# Autodesk Inventor assembly: BC-100000-Inf
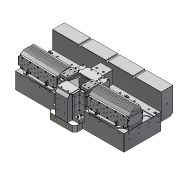
[picture p0: Inventor's stored thumbnail of the model, 180x180]
Saved by Autodesk Inventor 2016 (Build 200138000, 138)
## iProperties
Created: 2015-09-16
Part Number: BC-100000-Inf
Document SubType Name: Assembly
Designer: Reinaldo.Basílio
Mass: 576635 g
Surface Area: 46856.4 cm^2
Volume: 76554.8 cm^3
Density: 7.53231 g/cm^3
Author: Reinaldo.Basílio
## Documents named in this file (40)
- D:\ARQ\Basilio\LNLS-2\Anel\Dipolos\BC-3T\Dipolo 3T e 1T\Prototipo 1\Projeto Mecanico\BC-100000-Inf.iam
- D:\ARQ\Basilio\LNLS-2\Anel\Dipolos\BC-3T\Dipolo 3T e 1T\Prototipo 1\Projeto Mecanico\BC-100004.iam
- D:\ARQ\Basilio\LNLS-2\Anel\Dipolos\BC-3T\Dipolo 3T e 1T\Prototipo 1\Projeto Mecanico\BC-10005.ipt
- D:\ARQ\Basilio\LNLS-2\Anel\Dipolos\BC-3T\Dipolo 3T e 1T\Prototipo 1\Projeto Mecanico\BC-100005.iam
- D:\ARQ\Basilio\LNLS-2\Anel\Dipolos\BC-3T\Dipolo 3T e 1T\Prototipo 1\Projeto Mecanico\BC-10008.ipt
- D:\ARQ\Basilio\LNLS-2\Anel\Dipolos\BC-3T\Dipolo 3T e 1T\Prototipo 1\Projeto Mecanico\BC-10007.ipt
- D:\ARQ\Basilio\LNLS-2\Anel\Dipolos\BC-3T\Dipolo 3T e 1T\Prototipo 1\Projeto Mecanico\BC-10001.ipt
- D:\ARQ\Basilio\LNLS-2\Anel\Dipolos\BC-3T\Dipolo 3T e 1T\Prototipo 1\Projeto Mecanico\BC-10019-A.ipt
- D:\ARQ\Basilio\LNLS-2\Anel\Dipolos\BC-3T\Dipolo 3T e 1T\Prototipo 1\Projeto Mecanico\BC-100001-A-Inf.iam
- D:\ARQ\Basilio\LNLS-2\Anel\Dipolos\BC-3T\Dipolo 3T e 1T\Prototipo 1\Projeto Mecanico\BC-10002.ipt
- D:\ARQ\Basilio\LNLS-2\Anel\Dipolos\BC-3T\Dipolo 3T e 1T\Prototipo 1\Projeto Mecanico\BC-10006.ipt
- D:\ARQ\Basilio\LNLS-2\Anel\Dipolos\BC-3T\Dipolo 3T e 1T\Prototipo 1\Projeto Mecanico\BC-100001-B-Inf.iam
- D:\ARQ\Basilio\LNLS-2\Anel\Dipolos\BC-3T\Dipolo 3T e 1T\Prototipo 1\Projeto Mecanico\BC-10011.ipt
- D:\ARQ\Basilio\LNLS-2\Anel\Dipolos\BC-3T\Dipolo 3T e 1T\Prototipo 1\Projeto Mecanico\BC-10012.ipt
- D:\ARQ\Basilio\LNLS-2\Anel\Dipolos\BC-3T\Dipolo 3T e 1T\Prototipo 1\Projeto Mecanico\BC-10013.ipt
- D:\ARQ\Basilio\LNLS-2\Anel\Dipolos\BC-3T\Dipolo 3T e 1T\Prototipo 1\Projeto Mecanico\BC-10014.ipt
- D:\ARQ\Basilio\LNLS-2\Anel\Dipolos\BC-3T\Dipolo 3T e 1T\Prototipo 1\Projeto Mecanico\BC-10019-B.ipt
- D:\ARQ\Basilio\LNLS-2\Anel\Dipolos\BC-3T\Dipolo 3T e 1T\Prototipo 1\Projeto Mecanico\BC-10015.ipt
- D:\ARQ\Basilio\LNLS-2\Anel\Dipolos\BC-3T\Dipolo 3T e 1T\Prototipo 1\Projeto Mecanico\BC-10016.ipt
- D:\ARQ\Basilio\LNLS-2\Anel\Dipolos\BC-3T\Dipolo 3T e 1T\Prototipo 1\Projeto Mecanico\BC-10021.ipt
- D:\ARQ\Basilio\LNLS-2\Anel\Dipolos\BC-3T\Dipolo 3T e 1T\Prototipo 1\Projeto Mecanico\BC-10022.ipt
- D:\ARQ\Basilio\LNLS-2\Anel\Dipolos\BC-3T\Dipolo 3T e 1T\Prototipo 1\Projeto Mecanico\BC-10023.ipt
- D:\ARQ\Basilio\LNLS-2\Anel\Dipolos\BC-3T\Dipolo 3T e 1T\Prototipo 1\Projeto Mecanico\BC-10025.ipt
- D:\ARQ\Basilio\LNLS-2\Anel\Dipolos\BC-3T\Dipolo 3T e 1T\Prototipo 1\Projeto Mecanico\BC-10020.ipt
- D:\ARQ\Basilio\LNLS-2\Anel\Dipolos\BC-3T\Dipolo 3T e 1T\Prototipo 1\Projeto Mecanico\Parafusos\DIN 912 - M8x30.ipt
- D:\ARQ\Basilio\LNLS-2\Anel\Dipolos\BC-3T\Dipolo 3T e 1T\Prototipo 1\Projeto Mecanico\Parafusos\DIN 912 - M12x65.ipt
- D:\ARQ\Basilio\LNLS-2\Anel\Dipolos\BC-3T\Dipolo 3T e 1T\Prototipo 1\Projeto Mecanico\Parafusos\DIN 912 - M8x80.ipt
- D:\ARQ\Basilio\LNLS-2\Anel\Dipolos\BC-3T\Dipolo 3T e 1T\Prototipo 1\Projeto Mecanico\Parafusos\DIN 912 - M10x50.ipt
- D:\ARQ\Basilio\LNLS-2\Anel\Dipolos\BC-3T\Dipolo 3T e 1T\Prototipo 1\Projeto Mecanico\Parafusos\DIN 912 - M4x12.ipt
- D:\ARQ\Basilio\LNLS-2\Anel\Dipolos\BC-3T\Dipolo 3T e 1T\Prototipo 1\Projeto Mecanico\Parafusos\DIN 912 - M5x16.ipt
- D:\ARQ\Basilio\LNLS-2\Anel\Dipolos\BC-3T\Dipolo 3T e 1T\Prototipo 1\Projeto Mecanico\Parafusos\DIN 7991 - M5x12.ipt
- D:\ARQ\Basilio\LNLS-2\Anel\Dipolos\BC-3T\Dipolo 3T e 1T\Prototipo 1\Projeto Mecanico\Parafusos\DIN 125 - A 10,5.ipt
- D:\ARQ\Basilio\LNLS-2\Anel\Dipolos\BC-3T\Dipolo 3T e 1T\Prototipo 1\Projeto Mecanico\Parafusos\DIN 912 - M10x40.ipt
- D:\ARQ\Basilio\LNLS-2\Anel\Dipolos\BC-3T\Dipolo 3T e 1T\Prototipo 1\Projeto Mecanico\Parafusos\DIN 912 - M8x20.ipt
- D:\ARQ\Basilio\LNLS-2\Anel\Dipolos\BC-3T\Dipolo 3T e 1T\Prototipo 1\Projeto Mecanico\Parafusos\DIN 912 - M8x40.ipt
- D:\ARQ\Basilio\LNLS-2\Anel\Dipolos\BC-3T\Dipolo 3T e 1T\Prototipo 1\Projeto Mecanico\Parafusos\DIN 933 - M4x14.ipt
- D:\ARQ\Basilio\LNLS-2\Anel\Dipolos\BC-3T\Dipolo 3T e 1T\Prototipo 1\Projeto Mecanico\Parafusos\DIN 912 - M4x18.ipt
- D:\ARQ\Basilio\LNLS-2\Anel\Dipolos\BC-3T\Dipolo 3T e 1T\Prototipo 1\Projeto Mecanico\BC-10026.ipt
- D:\ARQ\Basilio\LNLS-2\Anel\Dipolos\BC-3T\Dipolo 3T e 1T\Prototipo 1\Projeto Mecanico\BC-10027.ipt
- D:\ARQ\Basilio\LNLS-2\Anel\Dipolos\BC-3T\Dipolo 3T e 1T\Prototipo 1\Projeto Mecanico\BC-100001\AIP\FEA\bjj5sjykh.fres
## Components (140 placed, 38 different names)
1. BC-10001:1 — Flush:41, Mate:39, Mate:48, Mate:50, Mate:52, Flush:57, Insert:3, Mate:53, Insert:6, Insert:7, Insert:8, Mate:54, Mate:55, Insert:13, Insert:15, Insert:16, Insert:22, Insert:23, Insert:24, Insert:25, Insert:26, Insert:27, Mate:57, Mate:62, Insert:30, Insert:31, Insert:48, Insert:49, Insert:50, Insert:51, Insert:52, Insert:53, Insert:54, Insert:55, Insert:56, Insert:57, Insert:58, Insert:59, Insert:154, Insert:155
2. BC-10002:1 — Flush:46, Mate:48, Mate:49, Insert:17, Insert:18, Insert:19, Insert:20, Insert:36, Insert:37, Insert:76, Insert:77
3. BC-10006:1 — Mate:52, Flush:57, Flush:58, Insert:68, Insert:69, Insert:70, Insert:71, Insert:72, Insert:73, Insert:74, Insert:75
4. BC-100005:1 [sub-assembly] — Flush:28, Mate:30, Flush:35, Mate:49, Mate:53
5. BC-100004:1 [sub-assembly] — Flush:24, Mate:17, Flush:25, Flush:26, Mate:50
6. BC-10019-B:1 — Insert:13, Insert:14, Insert:118, Insert:119, Insert:120, Insert:121
7. BC-10019-A:1 — Mate:39, Mate:40, Mate:41, Insert:110, Insert:111, Insert:112, Insert:113
8. BC-10005:1 — Mate:17, Flush:25, Flush:26, Mate:18, Flush:27, Flush:28, Mate:22, Flush:29, Mate:24, Flush:30, Mate:28, Flush:33, Mate:29, Flush:34, Mate:30, Flush:41, Mate:40, Mate:41, Flush:46, Insert:14
9. BC-100004:2 [sub-assembly] — Mate:22, Flush:29, Flush:31, Mate:59
10. BC-100004:3 [sub-assembly] — Mate:24, Flush:30, Flush:32, Flush:35, Mate:60
11. BC-100005:2 [sub-assembly] — Mate:18, Flush:27, Flush:31, Flush:32, Flush:34, Mate:61
12. BC-10008:1 — Insert:28, Insert:29, Insert:30, Insert:31, Insert:82, Insert:83, Insert:84, Insert:85
13. BC-10007:1 — Insert:28, Insert:29
14. BC-100001-A-Inf:1 [sub-assembly] — Insert:3, Tangent:2, Mate:54, Mate:63, Mate:64, Mate:65, Mate:66
15. BC-100001-B-Inf:1 [sub-assembly] — Insert:6, Tangent:1, Mate:55, Mate:67, Mate:68, Mate:69, Mate:70
16. BC-10011:1 — Insert:8, Tangent:1, Insert:145
17. BC-10011:2 — Insert:7, Tangent:2, Insert:144
18. BC-10012:1 — Insert:15, Insert:16, Insert:136, Insert:137
19. BC-10014:1 — Insert:17, Insert:18, Insert:126, Insert:127, Insert:128, Insert:129, Insert:130
20. BC-10013:1 — Insert:19, Insert:20, Insert:131, Insert:132, Insert:133, Insert:134, Insert:135
21. BC-10012:2 — Insert:22, Insert:23, Mate:58, Insert:138, Insert:139
22. BC-10015:1 — Insert:24, Insert:25, Insert:47, Insert:78, Insert:79
23. BC-10015:2 — Insert:26, Insert:27, Insert:45, Insert:80, Insert:81
24. BC-10016:1 — Mate:57, Mate:58, Mate:59, Insert:46, Insert:140, Insert:141
25. BC-10016:2 — Mate:60, Mate:61, Mate:62, Insert:44, Insert:142, Insert:143
26. BC-10021:1 — Insert:36, Insert:37, Insert:39, Insert:41, Insert:42, Insert:43, Insert:90, Insert:91, Insert:92, Insert:93, Insert:94, Insert:95, Insert:96, Insert:97, Insert:98, Insert:99, Insert:100, Insert:101, Insert:156, Insert:157, Insert:158, Insert:159
27. BC-10022:1 — Insert:41, Insert:42, Insert:146, Insert:147, Insert:148, Insert:149
28. BC-10022:2 — Insert:39, Insert:43, Insert:150, Insert:151, Insert:152, Insert:153
29. BC-10023:1 — Insert:44, Insert:45, Insert:106, Insert:107, Insert:108, Insert:109
30. BC-10023:2 — Insert:46, Insert:47, Insert:102, Insert:103, Insert:104, Insert:105
31. BC-10025:1 — Insert:48, Insert:89
32. BC-10025:2 — Insert:49, Insert:88
33. BC-10025:3 — Insert:50, Insert:87
34. BC-10025:4 — Insert:51, Insert:86
35. BC-10020:1 — Mate:65, Insert:52, Insert:61
36. BC-10020:2 — Mate:66, Insert:53, Insert:60
37. BC-10020:3 — Mate:63, Insert:54, Insert:63
38. BC-10020:4 — Mate:64, Insert:55, Insert:62
39. BC-10020:5 — Mate:67, Insert:58, Insert:66
40. BC-10020:6 — Mate:68, Insert:59, Insert:67
41. BC-10020:7 — Mate:69, Insert:56, Insert:65
42. BC-10020:8 — Mate:70, Insert:57, Insert:64
43. DIN 912 - Parafuso Allen com cabeça (Inox) M8x30:1 — Insert:60
44. DIN 912 - Parafuso Allen com cabeça (Inox) M8x30:2 — Insert:61
45. DIN 912 - Parafuso Allen com cabeça (Inox) M8x30:3 — Insert:63
46. DIN 912 - Parafuso Allen com cabeça (Inox) M8x30:4 — Insert:62
47. DIN 912 - Parafuso Allen com cabeça (Inox) M8x30:5 — Insert:66
48. DIN 912 - Parafuso Allen com cabeça (Inox) M8x30:6 — Insert:67
49. DIN 912 - Parafuso Allen com cabeça (Inox) M8x30:7 — Insert:65
50. DIN 912 - Parafuso Allen com cabeça (Inox) M8x30:8 — Insert:64
51. DIN 912 - Parafuso Allen com cabeça (inox) M12x65:1 — Insert:68
52. DIN 912 - Parafuso Allen com cabeça (inox) M12x65:2 — Insert:69
53. DIN 912 - Parafuso Allen com cabeça (inox) M12x65:3 — Insert:70
54. DIN 912 - Parafuso Allen com cabeça (inox) M12x65:4 — Insert:71
55. DIN 912 - Parafuso Allen com cabeça (inox) M12x65:5 — Insert:72
56. DIN 912 - Parafuso Allen com cabeça (inox) M12x65:6 — Insert:73
57. DIN 912 - Parafuso Allen com cabeça (inox) M12x65:7 — Insert:74
58. DIN 912 - Parafuso Allen com cabeça (inox) M12x65:8 — Insert:75
59. DIN 912 - Parafuso Allen com cabeça (inox) M8x80:1 — Insert:77
60. DIN 912 - Parafuso Allen com cabeça (inox) M8x80:2 — Insert:76
61. DIN 912 - Parafuso Allen com cabeça (inox) M8x80:3 — Insert:78
62. DIN 912 - Parafuso Allen com cabeça (inox) M8x80:4 — Insert:79
63. DIN 912 - Parafuso Allen com cabeça (inox) M8x80:5 — Insert:80
64. DIN 912 - Parafuso Allen com cabeça (inox) M8x80:6 — Insert:81
65. DIN 912 - Parafuso Allen com cabeça (inox) M10x50:1 — Insert:82
66. DIN 912 - Parafuso Allen com cabeça (inox) M10x50:2 — Insert:83
67. DIN 912 - Parafuso Allen com cabeça (inox) M10x50:3 — Insert:84
68. DIN 912 - Parafuso Allen com cabeça (inox) M10x50:4 — Insert:85
69. DIN 912 - Aço Inox M4x12:1 — Insert:86
70. DIN 912 - Aço Inox M4x12:2 — Insert:87
71. DIN 912 - Aço Inox M4x12:3 — Insert:88
72. DIN 912 - Aço Inox M4x12:4 — Insert:89
73. DIN 912 - Aço Inox M5x16:1 — Insert:90
74. DIN 912 - Aço Inox M5x16:2 — Insert:91
75. DIN 912 - Aço Inox M5x16:3 — Insert:92
76. DIN 912 - Aço Inox M5x16:4 — Insert:93
77. DIN 912 - Aço Inox M5x16:5 — Insert:94
78. DIN 912 - Aço Inox M5x16:6 — Insert:95
79. DIN 912 - Aço Inox M5x16:7 — Insert:96
80. DIN 912 - Aço Inox M5x16:8 — Insert:97
81. DIN 7991 - Parafuso Allen com cabeça chata (inox) M5x12:1 — Insert:98
82. DIN 7991 - Parafuso Allen com cabeça chata (inox) M5x12:2 — Insert:99
83. DIN 7991 - Parafuso Allen com cabeça chata (inox) M5x12:3 — Insert:100
84. DIN 7991 - Parafuso Allen com cabeça chata (inox) M5x12:4 — Insert:101
85. DIN 7991 - Parafuso Allen com cabeça chata (inox) M5x12:5 — Insert:104
86. DIN 7991 - Parafuso Allen com cabeça chata (inox) M5x12:6 — Insert:102
87. DIN 7991 - Parafuso Allen com cabeça chata (inox) M5x12:7 — Insert:105
88. DIN 7991 - Parafuso Allen com cabeça chata (inox) M5x12:8 — Insert:103
89. DIN 7991 - Parafuso Allen com cabeça chata (inox) M5x12:9 — Insert:106
90. DIN 7991 - Parafuso Allen com cabeça chata (inox) M5x12:10 — Insert:107
91. DIN 7991 - Parafuso Allen com cabeça chata (inox) M5x12:11 — Insert:109
92. DIN 7991 - Parafuso Allen com cabeça chata (inox) M5x12:12 — Insert:108
93. DIN 125 A - Aço Inox 316 A 10,5:1 — Insert:113, Insert:115
94. DIN 125 A - Aço Inox 316 A 10,5:2 — Insert:112, Insert:114
95. DIN 125 A - Aço Inox 316 A 10,5:3 — Insert:110, Insert:116
96. DIN 125 A - Aço Inox 316 A 10,5:4 — Insert:111, Insert:117
97. DIN 912 - Parafuso Allen com cabeça (inox) M10x40:1 — Insert:114
98. DIN 912 - Parafuso Allen com cabeça (inox) M10x40:2 — Insert:115
99. DIN 912 - Parafuso Allen com cabeça (inox) M10x40:3 — Insert:116
100. DIN 912 - Parafuso Allen com cabeça (inox) M10x40:4 — Insert:117
101. DIN 125 A - Aço Inox 316 A 10,5:5 — Insert:118, Insert:122
102. DIN 125 A - Aço Inox 316 A 10,5:6 — Insert:119, Insert:123
103. DIN 125 A - Aço Inox 316 A 10,5:7 — Insert:120, Insert:124
104. DIN 125 A - Aço Inox 316 A 10,5:8 — Insert:121, Insert:125
105. DIN 912 - Parafuso Allen com cabeça (inox) M10x40:5 — Insert:122
106. DIN 912 - Parafuso Allen com cabeça (inox) M10x40:6 — Insert:123
107. DIN 912 - Parafuso Allen com cabeça (inox) M10x40:7 — Insert:124
108. DIN 912 - Parafuso Allen com cabeça (inox) M10x40:8 — Insert:125
109. DIN 912 - Parafuso Allen com cabeça (Inox) M8x20:1 — Insert:126
110. DIN 912 - Parafuso Allen com cabeça (Inox) M8x20:2 — Insert:127
111. DIN 912 - Parafuso Allen com cabeça (Inox) M8x20:3 — Insert:128
112. DIN 912 - Parafuso Allen com cabeça (Inox) M8x20:4 — Insert:129
113. DIN 912 - Parafuso Allen com cabeça (Inox) M8x20:5 — Insert:130
114. DIN 912 - Parafuso Allen com cabeça (Inox) M8x20:6 — Insert:131
115. DIN 912 - Parafuso Allen com cabeça (Inox) M8x20:7 — Insert:132
116. DIN 912 - Parafuso Allen com cabeça (Inox) M8x20:8 — Insert:133
117. DIN 912 - Parafuso Allen com cabeça (Inox) M8x20:9 — Insert:134
118. DIN 912 - Parafuso Allen com cabeça (Inox) M8x20:10 — Insert:135
119. DIN 912 - Parafuso Allen com cabeça (Inox) M8x30:9 — Insert:136
120. DIN 912 - Parafuso Allen com cabeça (Inox) M8x30:10 — Insert:137
121. DIN 912 - Parafuso Allen com cabeça (Inox) M8x30:11 — Insert:138
122. DIN 912 - Parafuso Allen com cabeça (Inox) M8x30:12 — Insert:139
123. DIN 912 - Parafuso Allen com cabeça (Inox) M8x40:1 — Insert:140
124. DIN 912 - Parafuso Allen com cabeça (Inox) M8x40:2 — Insert:141
125. DIN 912 - Parafuso Allen com cabeça (Inox) M8x40:3 — Insert:142
126. DIN 912 - Parafuso Allen com cabeça (Inox) M8x40:4 — Insert:143
127. DIN 933 - Parafuso sextavado com rosca total  M4x20:1 — Insert:144
128. DIN 933 - Parafuso sextavado com rosca total  M4x20:2 — Insert:145
129. DIN 912 - Aço Inox M4x18:1 — Insert:146
130. DIN 912 - Aço Inox M4x18:2 — Insert:147
131. DIN 912 - Aço Inox M4x18:3 — Insert:148
132. DIN 912 - Aço Inox M4x18:4 — Insert:149
133. DIN 912 - Aço Inox M4x18:5 — Insert:150
134. DIN 912 - Aço Inox M4x18:6 — Insert:151
135. DIN 912 - Aço Inox M4x18:7 — Insert:152
136. DIN 912 - Aço Inox M4x18:8 — Insert:153
137. BC-10026:1 — Insert:154
138. BC-10026:2 — Insert:155
139. BC-10027:1 — Insert:156, Insert:157
140. BC-10027:2 — Insert:158, Insert:159
## Relationships (193: Insert 144, Mate 31, Flush 16, Tangent 2)
- Flush:24: BC-100004:1
- Mate:17: BC-100004:1 ↔ BC-10005:1
- Flush:25: BC-100004:1 ↔ BC-10005:1
- Flush:26: BC-100004:1 ↔ BC-10005:1
- Mate:18: BC-10005:1 ↔ BC-100005:2
- Flush:27: BC-10005:1 ↔ BC-100005:2
- Flush:28: BC-100005:1 ↔ BC-10005:1
- Mate:22: BC-10005:1 ↔ BC-100004:2
- Flush:29: BC-10005:1 ↔ BC-100004:2
- Mate:24: BC-10005:1 ↔ BC-100004:3
- Flush:30: BC-10005:1 ↔ BC-100004:3
- Flush:31: BC-100004:2 ↔ BC-100005:2
- Flush:32: BC-100004:3 ↔ BC-100005:2
- Mate:28: BC-10005:1
- Flush:33: BC-10005:1
- Mate:29: BC-10005:1
- Flush:34 (-30 mm): BC-10005:1 ↔ BC-100005:2
- Mate:30: BC-100005:1 ↔ BC-10005:1
- Flush:35: BC-100005:1 ↔ BC-100004:3
- Flush:41: BC-10001:1 ↔ BC-10005:1
- Mate:39: BC-10001:1 ↔ BC-10019-A:1
- Mate:40: BC-10019-A:1 ↔ BC-10005:1
- Mate:41: BC-10019-A:1 ↔ BC-10005:1
- Flush:46: BC-10002:1 ↔ BC-10005:1
- Mate:48: BC-10001:1 ↔ BC-10002:1
- Mate:49: BC-10002:1 ↔ BC-100005:1
- Mate:50: BC-10001:1 ↔ BC-100004:1
- Mate:52: BC-10001:1 ↔ BC-10006:1
- Flush:57: BC-10001:1 ↔ BC-10006:1
- Insert:3: BC-10001:1 ↔ BC-100001-A-Inf:1
- Flush:58: BC-10006:1
- Mate:53: BC-10001:1 ↔ BC-100005:1
- Insert:6: BC-10001:1 ↔ BC-100001-B-Inf:1
- Insert:7: BC-10001:1 ↔ BC-10011:2
- Insert:8: BC-10001:1 ↔ BC-10011:1
- Tangent:1: BC-100001-B-Inf:1 ↔ BC-10011:1
- Tangent:2: BC-100001-A-Inf:1 ↔ BC-10011:2
- Mate:54: BC-10001:1 ↔ BC-100001-A-Inf:1
- Mate:55: BC-10001:1 ↔ BC-100001-B-Inf:1
- Insert:13: BC-10001:1 ↔ BC-10019-B:1
- Insert:14: BC-10019-B:1 ↔ BC-10005:1
- Insert:15: BC-10001:1 ↔ BC-10012:1
- Insert:16: BC-10001:1 ↔ BC-10012:1
- Insert:17: BC-10002:1 ↔ BC-10014:1
- Insert:18: BC-10002:1 ↔ BC-10014:1
- Insert:19: BC-10002:1 ↔ BC-10013:1
- Insert:20: BC-10002:1 ↔ BC-10013:1
- Insert:22: BC-10001:1 ↔ BC-10012:2
- Insert:23: BC-10001:1 ↔ BC-10012:2
- Insert:24: BC-10001:1 ↔ BC-10015:1
- Insert:25: BC-10001:1 ↔ BC-10015:1
- Insert:26: BC-10001:1 ↔ BC-10015:2
- Insert:27: BC-10001:1 ↔ BC-10015:2
- Mate:57: BC-10001:1 ↔ BC-10016:1
- Mate:58: BC-10012:2 ↔ BC-10016:1
- Mate:59: BC-100004:2 ↔ BC-10016:1
- Mate:60: BC-100004:3 ↔ BC-10016:2
- Mate:61: BC-100005:2 ↔ BC-10016:2
- Mate:62: BC-10001:1 ↔ BC-10016:2
- Insert:28: BC-10008:1 ↔ BC-10007:1
- Insert:29: BC-10008:1 ↔ BC-10007:1
- Insert:30: BC-10001:1 ↔ BC-10008:1
- Insert:31: BC-10001:1 ↔ BC-10008:1
- Insert:36: BC-10002:1 ↔ BC-10021:1
- Insert:37: BC-10002:1 ↔ BC-10021:1
- Insert:39 (2.6 mm): BC-10021:1 ↔ BC-10022:2
- Insert:41 (2.6 mm): BC-10021:1 ↔ BC-10022:1
- Insert:42 (2.6 mm): BC-10021:1 ↔ BC-10022:1
- Insert:43 (2.6 mm): BC-10021:1 ↔ BC-10022:2
- Insert:44: BC-10016:2 ↔ BC-10023:1
- Insert:45: BC-10015:2 ↔ BC-10023:1
- Insert:46: BC-10016:1 ↔ BC-10023:2
- Insert:47: BC-10015:1 ↔ BC-10023:2
- Insert:48: BC-10001:1 ↔ BC-10025:1
- Insert:49: BC-10001:1 ↔ BC-10025:2
- Insert:50: BC-10001:1 ↔ BC-10025:3
- Insert:51: BC-10001:1 ↔ BC-10025:4
- Mate:63: BC-100001-A-Inf:1 ↔ BC-10020:3
- Mate:64: BC-100001-A-Inf:1 ↔ BC-10020:4
- Mate:65: BC-100001-A-Inf:1 ↔ BC-10020:1
- Mate:66: BC-100001-A-Inf:1 ↔ BC-10020:2
- Insert:52: BC-10001:1 ↔ BC-10020:1
- Insert:53: BC-10001:1 ↔ BC-10020:2
- Insert:54: BC-10001:1 ↔ BC-10020:3
- Insert:55: BC-10001:1 ↔ BC-10020:4
- Mate:67: BC-100001-B-Inf:1 ↔ BC-10020:5
- Mate:68: BC-100001-B-Inf:1 ↔ BC-10020:6
- Mate:69: BC-100001-B-Inf:1 ↔ BC-10020:7
- Mate:70: BC-100001-B-Inf:1 ↔ BC-10020:8
- Insert:56: BC-10001:1 ↔ BC-10020:7
- Insert:57: BC-10001:1 ↔ BC-10020:8
- Insert:58: BC-10001:1 ↔ BC-10020:5
- Insert:59: BC-10001:1 ↔ BC-10020:6
- Insert:60: BC-10020:2 ↔ DIN 912 - Parafuso Allen com cabeça (Inox) M8x30:1
- Insert:61: BC-10020:1 ↔ DIN 912 - Parafuso Allen com cabeça (Inox) M8x30:2
- Insert:62: BC-10020:4 ↔ DIN 912 - Parafuso Allen com cabeça (Inox) M8x30:4
- Insert:63: BC-10020:3 ↔ DIN 912 - Parafuso Allen com cabeça (Inox) M8x30:3
- Insert:64: BC-10020:8 ↔ DIN 912 - Parafuso Allen com cabeça (Inox) M8x30:8
- Insert:65: BC-10020:7 ↔ DIN 912 - Parafuso Allen com cabeça (Inox) M8x30:7
- Insert:66: BC-10020:5 ↔ DIN 912 - Parafuso Allen com cabeça (Inox) M8x30:5
- Insert:67: BC-10020:6 ↔ DIN 912 - Parafuso Allen com cabeça (Inox) M8x30:6
- Insert:68: BC-10006:1 ↔ DIN 912 - Parafuso Allen com cabeça (inox) M12x65:1
- Insert:69: BC-10006:1 ↔ DIN 912 - Parafuso Allen com cabeça (inox) M12x65:2
- Insert:70: BC-10006:1 ↔ DIN 912 - Parafuso Allen com cabeça (inox) M12x65:3
- Insert:71: BC-10006:1 ↔ DIN 912 - Parafuso Allen com cabeça (inox) M12x65:4
- Insert:72: BC-10006:1 ↔ DIN 912 - Parafuso Allen com cabeça (inox) M12x65:5
- Insert:73: BC-10006:1 ↔ DIN 912 - Parafuso Allen com cabeça (inox) M12x65:6
- Insert:74: BC-10006:1 ↔ DIN 912 - Parafuso Allen com cabeça (inox) M12x65:7
- Insert:75: BC-10006:1 ↔ DIN 912 - Parafuso Allen com cabeça (inox) M12x65:8
- Insert:76: BC-10002:1 ↔ DIN 912 - Parafuso Allen com cabeça (inox) M8x80:2
- Insert:77: BC-10002:1 ↔ DIN 912 - Parafuso Allen com cabeça (inox) M8x80:1
- Insert:78: BC-10015:1 ↔ DIN 912 - Parafuso Allen com cabeça (inox) M8x80:3
- Insert:79: BC-10015:1 ↔ DIN 912 - Parafuso Allen com cabeça (inox) M8x80:4
- Insert:80: BC-10015:2 ↔ DIN 912 - Parafuso Allen com cabeça (inox) M8x80:5
- Insert:81: BC-10015:2 ↔ DIN 912 - Parafuso Allen com cabeça (inox) M8x80:6
- Insert:82: BC-10008:1 ↔ DIN 912 - Parafuso Allen com cabeça (inox) M10x50:1
- Insert:83: BC-10008:1 ↔ DIN 912 - Parafuso Allen com cabeça (inox) M10x50:2
- Insert:84: BC-10008:1 ↔ DIN 912 - Parafuso Allen com cabeça (inox) M10x50:3
- Insert:85: BC-10008:1 ↔ DIN 912 - Parafuso Allen com cabeça (inox) M10x50:4
- Insert:86: BC-10025:4 ↔ DIN 912 - Aço Inox M4x12:1
- Insert:87: BC-10025:3 ↔ DIN 912 - Aço Inox M4x12:2
- Insert:88: BC-10025:2 ↔ DIN 912 - Aço Inox M4x12:3
- Insert:89: BC-10025:1 ↔ DIN 912 - Aço Inox M4x12:4
- Insert:90: BC-10021:1 ↔ DIN 912 - Aço Inox M5x16:1
- Insert:91: BC-10021:1 ↔ DIN 912 - Aço Inox M5x16:2
- Insert:92: BC-10021:1 ↔ DIN 912 - Aço Inox M5x16:3
- Insert:93: BC-10021:1 ↔ DIN 912 - Aço Inox M5x16:4
- Insert:94: BC-10021:1 ↔ DIN 912 - Aço Inox M5x16:5
- Insert:95: BC-10021:1 ↔ DIN 912 - Aço Inox M5x16:6
- Insert:96: BC-10021:1 ↔ DIN 912 - Aço Inox M5x16:7
- Insert:97: BC-10021:1 ↔ DIN 912 - Aço Inox M5x16:8
- Insert:98: BC-10021:1 ↔ DIN 7991 - Parafuso Allen com cabeça chata (inox) M5x12:1
- Insert:99: BC-10021:1 ↔ DIN 7991 - Parafuso Allen com cabeça chata (inox) M5x12:2
- Insert:100: BC-10021:1 ↔ DIN 7991 - Parafuso Allen com cabeça chata (inox) M5x12:3
- Insert:101: BC-10021:1 ↔ DIN 7991 - Parafuso Allen com cabeça chata (inox) M5x12:4
- Insert:102: BC-10023:2 ↔ DIN 7991 - Parafuso Allen com cabeça chata (inox) M5x12:6
- Insert:103: BC-10023:2 ↔ DIN 7991 - Parafuso Allen com cabeça chata (inox) M5x12:8
- Insert:104: BC-10023:2 ↔ DIN 7991 - Parafuso Allen com cabeça chata (inox) M5x12:5
- Insert:105: BC-10023:2 ↔ DIN 7991 - Parafuso Allen com cabeça chata (inox) M5x12:7
- Insert:106: BC-10023:1 ↔ DIN 7991 - Parafuso Allen com cabeça chata (inox) M5x12:9
- Insert:107: BC-10023:1 ↔ DIN 7991 - Parafuso Allen com cabeça chata (inox) M5x12:10
- Insert:108: BC-10023:1 ↔ DIN 7991 - Parafuso Allen com cabeça chata (inox) M5x12:12
- Insert:109: BC-10023:1 ↔ DIN 7991 - Parafuso Allen com cabeça chata (inox) M5x12:11
- Insert:110: BC-10019-A:1 ↔ DIN 125 A - Aço Inox 316 A 10,5:3
- Insert:111: BC-10019-A:1 ↔ DIN 125 A - Aço Inox 316 A 10,5:4
- Insert:112: BC-10019-A:1 ↔ DIN 125 A - Aço Inox 316 A 10,5:2
- Insert:113: BC-10019-A:1 ↔ DIN 125 A - Aço Inox 316 A 10,5:1
- Insert:114: DIN 125 A - Aço Inox 316 A 10,5:2 ↔ DIN 912 - Parafuso Allen com cabeça (inox) M10x40:1
- Insert:115: DIN 125 A - Aço Inox 316 A 10,5:1 ↔ DIN 912 - Parafuso Allen com cabeça (inox) M10x40:2
- Insert:116: DIN 125 A - Aço Inox 316 A 10,5:3 ↔ DIN 912 - Parafuso Allen com cabeça (inox) M10x40:3
- Insert:117: DIN 125 A - Aço Inox 316 A 10,5:4 ↔ DIN 912 - Parafuso Allen com cabeça (inox) M10x40:4
- Insert:118: BC-10019-B:1 ↔ DIN 125 A - Aço Inox 316 A 10,5:5
- Insert:119: BC-10019-B:1 ↔ DIN 125 A - Aço Inox 316 A 10,5:6
- Insert:120: BC-10019-B:1 ↔ DIN 125 A - Aço Inox 316 A 10,5:7
- Insert:121: BC-10019-B:1 ↔ DIN 125 A - Aço Inox 316 A 10,5:8
- Insert:122: DIN 125 A - Aço Inox 316 A 10,5:5 ↔ DIN 912 - Parafuso Allen com cabeça (inox) M10x40:5
- Insert:123: DIN 125 A - Aço Inox 316 A 10,5:6 ↔ DIN 912 - Parafuso Allen com cabeça (inox) M10x40:6
- Insert:124: DIN 125 A - Aço Inox 316 A 10,5:7 ↔ DIN 912 - Parafuso Allen com cabeça (inox) M10x40:7
- Insert:125: DIN 125 A - Aço Inox 316 A 10,5:8 ↔ DIN 912 - Parafuso Allen com cabeça (inox) M10x40:8
- Insert:126: BC-10014:1 ↔ DIN 912 - Parafuso Allen com cabeça (Inox) M8x20:1
- Insert:127: BC-10014:1 ↔ DIN 912 - Parafuso Allen com cabeça (Inox) M8x20:2
- Insert:128: BC-10014:1 ↔ DIN 912 - Parafuso Allen com cabeça (Inox) M8x20:3
- Insert:129: BC-10014:1 ↔ DIN 912 - Parafuso Allen com cabeça (Inox) M8x20:4
- Insert:130: BC-10014:1 ↔ DIN 912 - Parafuso Allen com cabeça (Inox) M8x20:5
- Insert:131: BC-10013:1 ↔ DIN 912 - Parafuso Allen com cabeça (Inox) M8x20:6
- Insert:132: BC-10013:1 ↔ DIN 912 - Parafuso Allen com cabeça (Inox) M8x20:7
- Insert:133: BC-10013:1 ↔ DIN 912 - Parafuso Allen com cabeça (Inox) M8x20:8
- Insert:134: BC-10013:1 ↔ DIN 912 - Parafuso Allen com cabeça (Inox) M8x20:9
- Insert:135: BC-10013:1 ↔ DIN 912 - Parafuso Allen com cabeça (Inox) M8x20:10
- Insert:136: BC-10012:1 ↔ DIN 912 - Parafuso Allen com cabeça (Inox) M8x30:9
- Insert:137: BC-10012:1 ↔ DIN 912 - Parafuso Allen com cabeça (Inox) M8x30:10
- Insert:138: BC-10012:2 ↔ DIN 912 - Parafuso Allen com cabeça (Inox) M8x30:11
- Insert:139: BC-10012:2 ↔ DIN 912 - Parafuso Allen com cabeça (Inox) M8x30:12
- Insert:140: BC-10016:1 ↔ DIN 912 - Parafuso Allen com cabeça (Inox) M8x40:1
- Insert:141: BC-10016:1 ↔ DIN 912 - Parafuso Allen com cabeça (Inox) M8x40:2
- Insert:142: BC-10016:2 ↔ DIN 912 - Parafuso Allen com cabeça (Inox) M8x40:3
- Insert:143: BC-10016:2 ↔ DIN 912 - Parafuso Allen com cabeça (Inox) M8x40:4
- Insert:144: BC-10011:2 ↔ DIN 933 - Parafuso sextavado com rosca total  M4x20:1
- Insert:145: BC-10011:1 ↔ DIN 933 - Parafuso sextavado com rosca total  M4x20:2
- Insert:146: BC-10022:1 ↔ DIN 912 - Aço Inox M4x18:1
- Insert:147: BC-10022:1 ↔ DIN 912 - Aço Inox M4x18:2
- Insert:148: BC-10022:1 ↔ DIN 912 - Aço Inox M4x18:3
- Insert:149: BC-10022:1 ↔ DIN 912 - Aço Inox M4x18:4
- Insert:150: BC-10022:2 ↔ DIN 912 - Aço Inox M4x18:5
- Insert:151: BC-10022:2 ↔ DIN 912 - Aço Inox M4x18:6
- Insert:152: BC-10022:2 ↔ DIN 912 - Aço Inox M4x18:7
- Insert:153: BC-10022:2 ↔ DIN 912 - Aço Inox M4x18:8
- Insert:154: BC-10001:1 ↔ BC-10026:1
- Insert:155: BC-10001:1 ↔ BC-10026:2
- Insert:156: BC-10021:1 ↔ BC-10027:1
- Insert:157: BC-10021:1 ↔ BC-10027:1
- Insert:158: BC-10021:1 ↔ BC-10027:2
- Insert:159: BC-10021:1 ↔ BC-10027:2
